# Autodesk Inventor assembly: Ensamble tablero
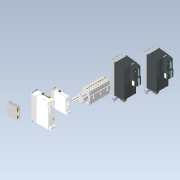
[picture p0: Inventor's stored thumbnail of the model, 180x180]
Saved by Autodesk Inventor 2021 (Build 250183000, 183)
## iProperties
Created: 2021-08-22
Part Number: Ensamble tablero
Document SubType Name: Assembly
Designer: Andrés Holguín
Author: Andrés Holguín
## Documents named in this file (9)
- C:\Users\andre\Documents\GitHub\Dis.-Mecatronico-E6\inventor proyecto\Tablero\Ensamble tablero.iam
- C:\Users\andre\Documents\GitHub\Dis.-Mecatronico-E6\inventor proyecto\Tablero\Interruptores\3p30.ipt
- C:\Users\andre\Documents\GitHub\Dis.-Mecatronico-E6\inventor proyecto\Tablero\Interruptores\3p50.ipt
- C:\Users\andre\Documents\GitHub\Dis.-Mecatronico-E6\inventor proyecto\Tablero\Interruptores\2p8\a9n18344.iam
- C:\Users\andre\Documents\GitHub\Dis.-Mecatronico-E6\inventor proyecto\Tablero\Riel DIN\Riel DIN.ipt
- C:\Users\andre\Documents\GitHub\Dis.-Mecatronico-E6\inventor proyecto\Tablero\Variador\G120_G120_3D_3654a134dd9c4e348126222df3348349.iam
- C:\Users\andre\Documents\GitHub\Dis.-Mecatronico-E6\inventor proyecto\Tablero\DriveAvance\PARTserver0202108230417182353949810e898ce\AIS2021\5340825 CMMT-AS-C4-3A-EP-S1.iam
- C:\Users\andre\Documents\GitHub\Dis.-Mecatronico-E6\inventor proyecto\Tablero\DriveActuador\AIS2021\8133356 CMMT-AS-C7-11A-P3-EP-S1.iam
- C:\Users\andre\Documents\GitHub\Dis.-Mecatronico-E6\inventor proyecto\Tablero\DriveActuador\2247681 CACN-3A-1-5.ipt
## Components (10 placed, 8 different names)
1. 3p30:1 — Rigid:2, Rigid:3
2. 3p50:2 — Rigid:1, Mate:1
3. 3p50:1 — Rigid:1, Rigid:2
4. a9n18344:1 [sub-assembly] — Rigid:3
5. Riel DIN:1 — Mate:1
6. G120_G120_3D_3654a134dd9c4e348126222df3348349:1 [sub-assembly]
7. G120_G120_3D_3654a134dd9c4e348126222df3348349:2 [sub-assembly]
8. 5340825 CMMT-AS-C4-3A-EP-S1:1 [sub-assembly]
9. 8133356 CMMT-AS-C7-11A-P3-EP-S1:1 [sub-assembly]
10. 2247681 CACN-3A-1-5:1
## Relationships (4: WeldJoint 3, Mate 1)
- Rigid:1 [WeldJoint]: 3p50:2 ↔ 3p50:1
- Rigid:2 [WeldJoint]: 3p30:1 ↔ 3p50:1
- Rigid:3 [WeldJoint]: 3p30:1 ↔ a9n18344:1
- Mate:1: 3p50:2 ↔ Riel DIN:1
